# Autodesk Inventor assembly: Шкив
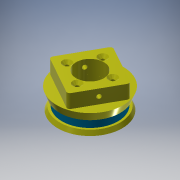
[picture p0: Inventor's stored thumbnail of the model, 180x180]
Saved by Autodesk Inventor 2019.1 (Build 231200000, 200)
## iProperties
Created: 2018-10-15
Part Number: Шкив
Material: Типовые
Document SubType Name: Assembly
Designer: Олег
Author: Олег
## Documents named in this file (5)
- C:\Users\Олег\OneDrive\Общая\NoSpace 2.0\Манипулятор\Шкив.iam
- C:\Users\Олег\OneDrive\Общая\NoSpace 2.0\Манипулятор\Крепление шкива с обратной стороны.ipt
- C:\Users\Олег\OneDrive\Общая\NoSpace 2.0\Манипулятор\Крепление шкива со стороны выступа.ipt
- C:\Users\Олег\OneDrive\Общая\NoSpace 2.0\Манипулятор\Фиксатор шкива на оси.ipt
- C:\Users\Олег\OneDrive\Общая\NoSpace 2.0\Манипулятор\Шкив mxl.ipt
## Components (4 placed, 4 different names)
1. Крепление шкива с обратной стороны:1 — Совмещение:6, Совмещение:7, Совмещение:8
2. Крепление шкива со стороны выступа:1 — Совмещение:1, Совмещение:3, Совмещение:4, Совмещение:5, Совмещение:9
3. Фиксатор шкива на оси:1 — Совмещение:3, Совмещение:4, Совмещение:5, Совмещение:7, Совмещение:8
4. Шкив mxl:1 — Совмещение:1, Совмещение:6, Совмещение:9
## Relationships (8: Mate 8)
- Совмещение:1 [Mate]: Крепление шкива со стороны выступа:1 ↔ Шкив mxl:1
- Совмещение:3 [Mate]: Крепление шкива со стороны выступа:1 ↔ Фиксатор шкива на оси:1
- Совмещение:4 [Mate]: Крепление шкива со стороны выступа:1 ↔ Фиксатор шкива на оси:1
- Совмещение:5 [Mate]: Крепление шкива со стороны выступа:1 ↔ Фиксатор шкива на оси:1
- Совмещение:6 [Mate]: Крепление шкива с обратной стороны:1 ↔ Шкив mxl:1
- Совмещение:7 [Mate]: Крепление шкива с обратной стороны:1 ↔ Фиксатор шкива на оси:1
- Совмещение:8 [Mate]: Крепление шкива с обратной стороны:1 ↔ Фиксатор шкива на оси:1
- Совмещение:9 [Mate]: Крепление шкива со стороны выступа:1 ↔ Шкив mxl:1
